# Autodesk Inventor assembly: Assembly1
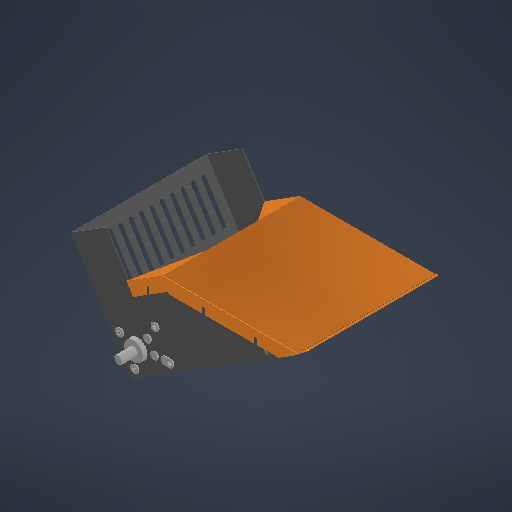
[picture p0: Inventor's stored thumbnail of the model, 512x512]
Saved by Autodesk Inventor 2026.2 (Build 302298000, 298)
## iProperties
Created: 2026-03-06
Part Number: Assembly1
Document SubType Name: Assembly
Designer: User
Author: User
## Documents named in this file (4)
- C:\Users\User\Documents\3D\robo sumo\Assembly1.iam
- C:\Users\User\Documents\3D\robo sumo\qveda_korpusi.ipt
- C:\Users\User\Documents\3D\robo sumo\5840-31ZY D8\5840-31ZY D8\5840-31ZY D8.ipt
- C:\Users\User\Documents\3D\robo sumo\kapoti.ipt
## Components (4 placed, 3 different names)
1. qveda_korpusi:1 — Mate:1, Mate:2, Mate:3, Mate:4, Mate:5, Mate:6, Mate:7, Mate:8, Mate:9
2. 5840-31ZY D8:1 — Mate:4, Mate:5, Mate:6
3. 5840-31ZY D8:2 — Mate:1, Mate:2, Mate:3
4. kapoti:1 — Mate:7, Mate:8, Mate:9
## Relationships (9: Mate 9)
- Mate:1: qveda_korpusi:1 ↔ 5840-31ZY D8:2
- Mate:2: qveda_korpusi:1 ↔ 5840-31ZY D8:2
- Mate:3: qveda_korpusi:1 ↔ 5840-31ZY D8:2
- Mate:4: qveda_korpusi:1 ↔ 5840-31ZY D8:1
- Mate:5: qveda_korpusi:1 ↔ 5840-31ZY D8:1
- Mate:6: qveda_korpusi:1 ↔ 5840-31ZY D8:1
- Mate:7: qveda_korpusi:1 ↔ kapoti:1
- Mate:8: qveda_korpusi:1 ↔ kapoti:1
- Mate:9: qveda_korpusi:1 ↔ kapoti:1
